# Autodesk Inventor assembly: arm-second
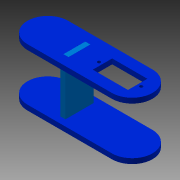
[picture p0: Inventor's stored thumbnail of the model, 180x180]
Saved by Autodesk Inventor 2013 (Build 170138000, 138)
## iProperties
Created: 2012-09-09
Part Number: arm-second
Document SubType Name: Assembly
Designer: frankenteddy
Author: frankenteddy
## Documents named in this file (4)
- C:\Users\frankenteddy\Desktop\oshawatt1\arm-second.iam
- C:\Users\frankenteddy\Desktop\oshawatt1\arm-second-back.ipt
- C:\Users\frankenteddy\Desktop\oshawatt1\arm-second-strut.ipt
- C:\Users\frankenteddy\Desktop\oshawatt1\arm-second-front.ipt
## Components (3 placed, 3 different names)
1. arm-second-back:1 — Mate:4, Mate:5, Mate:6
2. arm-second-strut:1 — Mate:1, Mate:2, Mate:3, Mate:4, Mate:5, Mate:6
3. arm-second-front:1 — Mate:1, Mate:2, Mate:3
## Relationships (6: Mate 6)
- Mate:1: arm-second-strut:1 ↔ arm-second-front:1
- Mate:2: arm-second-strut:1 ↔ arm-second-front:1
- Mate:3: arm-second-strut:1 ↔ arm-second-front:1
- Mate:4: arm-second-back:1 ↔ arm-second-strut:1
- Mate:5: arm-second-back:1 ↔ arm-second-strut:1
- Mate:6: arm-second-back:1 ↔ arm-second-strut:1
